# Autodesk Inventor assembly: Casing
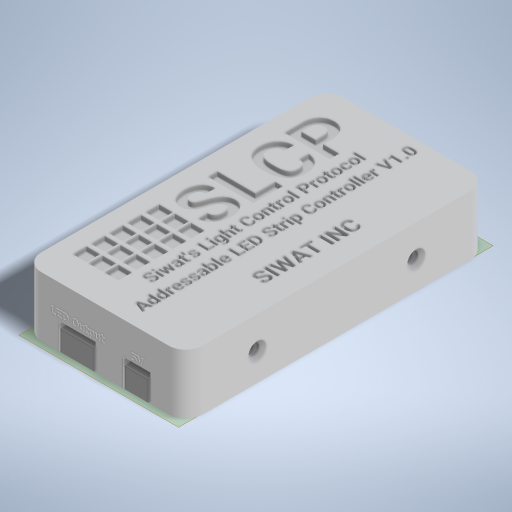
[picture p0: Inventor's stored thumbnail of the model, 512x512]
Saved by Autodesk Inventor 2023 (Build 270158000, 158)
## iProperties
Created: 2022-06-08
Part Number: Casing
Document SubType Name: Assembly
Designer: siwat
Author: siwat
## Documents named in this file (4)
- D:\Git\pi-pico-slcp-case\Casing.iam
- D:\Git\pi-pico-slcp-case\Base.ipt
- D:\Git\pi-pico-slcp-case\raspberry-pi-pico-r3-1.snapshot.1\Raspberry Pi Pico-R3.ipt
- D:\Git\pi-pico-slcp-case\cover.ipt
## Components (3 placed, 3 different names)
1. Base:1 — Flush:1, Flush:2
2. Raspberry Pi Pico-R3:1
3. cover:1 — Flush:1, Flush:2
## Relationships (2: Flush 2)
- Flush:1: Base:1 ↔ cover:1
- Flush:2: Base:1 ↔ cover:1
